# Autodesk Inventor assembly: untitled.brd
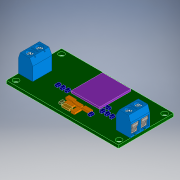
[picture p0: Inventor's stored thumbnail of the model, 180x180]
Saved by Autodesk Inventor 2022 (Build 260153000, 153)
## iProperties
Created: 2022-02-26
Part Number: untitled.brd
Document SubType Name: Assembly
Designer: Petrov Ivan
Author: Petrov Ivan
## Documents named in this file (8)
- D:\IVAN\Ivan_desktop\Kvantorium\Projects\YouBotRobot\electronic\jetson_power_board\untitled.brd.iam
- D:\IVAN\Ivan_desktop\Kvantorium\Projects\YouBotRobot\electronic\jetson_power_board\untitled.brdКонтур.ipt
- D:\IVAN\Ivan_desktop\Kvantorium\Projects\YouBotRobot\electronic\jetson_power_board\C0805K, C0805K_1.ipt
- D:\IVAN\Ivan_desktop\Kvantorium\Projects\YouBotRobot\electronic\jetson_power_board\SOD-123_MINI-SMA, CGRM4004-G_13.ipt
- D:\IVAN\Ivan_desktop\Kvantorium\Projects\YouBotRobot\electronic\jetson_power_board\CHIPLED_0805, CHIPLED_0805_19.ipt
- D:\IVAN\Ivan_desktop\Kvantorium\Projects\YouBotRobot\electronic\jetson_power_board\R0805, R0805_21.ipt
- D:\IVAN\Ivan_desktop\Kvantorium\Projects\YouBotRobot\electronic\jetson_power_board\LMZ13610, LMZ13610_27.ipt
- D:\IVAN\Ivan_desktop\Kvantorium\Projects\YouBotRobot\electronic\jetson_power_board\Terminal Block 2P.ipt
## Components (19 placed, 18 different names)
1. untitled.brdКонтур:1 — Совмещение:1, Касательность:1, Касательность:2, Угол:1, Совмещение:2, Совмещение:3, Угол:2
2. C1_2
3. C2_3
4. C3_4
5. C4_5
6. C5_6
7. C6_7
8. C7_8
9. C8_9
10. D1_14
11. LED1_20
12. R1_22
13. R2_23
14. R3_24
15. R4_25
16. R5_26
17. U_1_28
18. Terminal Block 2P:1 — Совмещение:1, Касательность:1, Касательность:2, Угол:1
19. Terminal Block 2P:2 — Совмещение:2, Совмещение:3, Угол:2
## Relationships (7: Mate 3, Tangent 2, Angle 2)
- Совмещение:1 [Mate]: untitled.brdКонтур:1 ↔ Terminal Block 2P:1
- Касательность:1 [Tangent]: untitled.brdКонтур:1 ↔ Terminal Block 2P:1
- Касательность:2 [Tangent]: untitled.brdКонтур:1 ↔ Terminal Block 2P:1
- Угол:1 [Angle] (0 deg): untitled.brdКонтур:1 ↔ Terminal Block 2P:1
- Совмещение:2 [Mate]: untitled.brdКонтур:1 ↔ Terminal Block 2P:2
- Совмещение:3 [Mate]: untitled.brdКонтур:1 ↔ Terminal Block 2P:2
- Угол:2 [Angle] (0 deg): untitled.brdКонтур:1 ↔ Terminal Block 2P:2
